# Autodesk Inventor assembly: SonarMount180
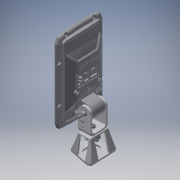
[picture p0: Inventor's stored thumbnail of the model, 180x180]
Saved by Autodesk Inventor 2018 (Build 220112000, 112)
## iProperties
Created: 2019-05-28
Part Number: SonarMount180
Document SubType Name: Assembly
Designer: Ash
Author: Ash
## Documents named in this file (9)
- C:\Autodesk\Skills 2019 Nationals\Competition\SonarMount180.iam
- C:\Autodesk\Skills 2019 Nationals\Competition\Back Plate.ipt
- C:\Autodesk\Skills 2019 Nationals\Competition\MountRotater.ipt
- C:\Autodesk\Skills 2019 Nationals\Competition\MainMount.ipt
- C:\Autodesk\Skills 2019 Nationals\Competition\Mounting Template.ipt
- C:\Autodesk\Skills 2019 Nationals\Competition\GivenFiles\Day 1 AM\Day 1 AM\Day 1 AM\98671A190_BLACK LUSTER STEEL AND IRON WING NUTS.ipt
- C:\Autodesk\Skills 2019 Nationals\Competition\GivenFiles\Day 1 AM\Day 1 AM\Day 1 AM\91251A342_BLACK-OXIDE ALLOY STEEL SOCKET HEAD CAP SCREW.ipt
- C:\Autodesk\Skills 2019 Nationals\Competition\GivenFiles\Day 1 AM\Day 1 AM\Day 1 AM\90044A120_BLACK-OXIDE ALLOY STEEL SOCKET HEAD CAP SCREW.ipt
- C:\Autodesk\Skills 2019 Nationals\Competition\GivenFiles\Day 1 AM\Day 1 AM\Day 1 AM\90107A011_TYPE 316 STAINLESS STEEL FLAT WASHER.ipt
## Components (12 placed, 8 different names)
1. Back Plate:1 — Mate:1, Mate:2, Angle:1, Mate:9
2. MountRotater:1 — Mate:1, Mate:3, Mate:6
3. MountRotater:2 — Mate:2, Mate:3, Mate:4, Mate:5
4. MainMount:1 — Mate:4, Mate:5, Mate:6, Angle:1, Mate:7, Mate:8, Mate:9, Mate:10, Mate:11, Mate:14, Mate:15, Mate:18, Mate:22, Angle:2
5. Mounting Template:1 — Mate:7, Mate:8, Mate:13, Mate:20, Angle:2
6. 98671A190_BLACK LUSTER STEEL AND IRON WING NUTS:1 — Mate:12, Mate:13
7. 98671A190_BLACK LUSTER STEEL AND IRON WING NUTS:2 — Mate:16, Mate:23
8. 91251A342_BLACK-OXIDE ALLOY STEEL SOCKET HEAD CAP SCREW:1 — Mate:10, Mate:11, Mate:12, Mate:17, Mate:19
9. 90044A120_BLACK-OXIDE ALLOY STEEL SOCKET HEAD CAP SCREW:1 — Mate:14, Mate:15, Mate:16, Mate:21
10. 90107A011_TYPE 316 STAINLESS STEEL FLAT WASHER:1 — Mate:21, Mate:22, Mate:23
11. 90107A011_TYPE 316 STAINLESS STEEL FLAT WASHER:2 — Mate:17, Mate:18
12. 90107A011_TYPE 316 STAINLESS STEEL FLAT WASHER:3 — Mate:19, Mate:20
## Relationships (25: Mate 23, Angle 2)
- Mate:1: Back Plate:1 ↔ MountRotater:1
- Mate:2: Back Plate:1 ↔ MountRotater:2
- Mate:3: MountRotater:1 ↔ MountRotater:2
- Mate:4: MountRotater:2 ↔ MainMount:1
- Mate:5: MountRotater:2 ↔ MainMount:1
- Mate:6: MountRotater:1 ↔ MainMount:1
- Angle:1 (0 deg): Back Plate:1 ↔ MainMount:1
- Mate:7: MainMount:1 ↔ Mounting Template:1
- Mate:8 (1.27 mm): MainMount:1 ↔ Mounting Template:1
- Mate:9 (3.175 mm): Back Plate:1 ↔ MainMount:1
- Mate:10: MainMount:1 ↔ 91251A342_BLACK-OXIDE ALLOY STEEL SOCKET HEAD CAP SCREW:1
- Mate:11: MainMount:1 ↔ 91251A342_BLACK-OXIDE ALLOY STEEL SOCKET HEAD CAP SCREW:1
- Mate:12: 98671A190_BLACK LUSTER STEEL AND IRON WING NUTS:1 ↔ 91251A342_BLACK-OXIDE ALLOY STEEL SOCKET HEAD CAP SCREW:1
- Mate:13: Mounting Template:1 ↔ 98671A190_BLACK LUSTER STEEL AND IRON WING NUTS:1
- Mate:14: MainMount:1 ↔ 90044A120_BLACK-OXIDE ALLOY STEEL SOCKET HEAD CAP SCREW:1
- Mate:15: MainMount:1 ↔ 90044A120_BLACK-OXIDE ALLOY STEEL SOCKET HEAD CAP SCREW:1
- Mate:16: 98671A190_BLACK LUSTER STEEL AND IRON WING NUTS:2 ↔ 90044A120_BLACK-OXIDE ALLOY STEEL SOCKET HEAD CAP SCREW:1
- Mate:17: 91251A342_BLACK-OXIDE ALLOY STEEL SOCKET HEAD CAP SCREW:1 ↔ 90107A011_TYPE 316 STAINLESS STEEL FLAT WASHER:2
- Mate:18: MainMount:1 ↔ 90107A011_TYPE 316 STAINLESS STEEL FLAT WASHER:2
- Mate:19: 91251A342_BLACK-OXIDE ALLOY STEEL SOCKET HEAD CAP SCREW:1 ↔ 90107A011_TYPE 316 STAINLESS STEEL FLAT WASHER:3
- Mate:20: Mounting Template:1 ↔ 90107A011_TYPE 316 STAINLESS STEEL FLAT WASHER:3
- Mate:21: 90044A120_BLACK-OXIDE ALLOY STEEL SOCKET HEAD CAP SCREW:1 ↔ 90107A011_TYPE 316 STAINLESS STEEL FLAT WASHER:1
- Mate:22: MainMount:1 ↔ 90107A011_TYPE 316 STAINLESS STEEL FLAT WASHER:1
- Mate:23: 98671A190_BLACK LUSTER STEEL AND IRON WING NUTS:2 ↔ 90107A011_TYPE 316 STAINLESS STEEL FLAT WASHER:1
- Angle:2 (180 deg): MainMount:1 ↔ Mounting Template:1
